# Autodesk Inventor assembly: PendulumAssembly
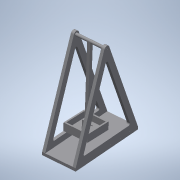
[picture p0: Inventor's stored thumbnail of the model, 180x180]
Saved by Autodesk Inventor 2020 (Build 240168000, 168)
## iProperties
Created: 2020-04-07
Part Number: PendulumAssembly
Document SubType Name: Assembly
Designer: gman
Author: gman
## Documents named in this file (5)
- C:\Users\gman\Desktop\CAD\Physics\PendulumAssembly.iam
- C:\Users\gman\Desktop\CAD\Physics\Outside.ipt
- C:\Users\gman\Desktop\CAD\Physics\PendulumHanger.ipt
- C:\Users\gman\Desktop\CAD\Physics\Base.ipt
- C:\Users\gman\Desktop\CAD\Physics\WeightBasket.ipt
## Components (5 placed, 4 different names)
1. Base:1 — Mate:1, Flush:1, Mate:2, Mate:3, Mate:4, Flush:2, Mate:8
2. Outside:1 — Mate:4, Flush:2, Rotational:1, Mate:8
3. Outside:2 — Flush:1, Mate:2, Mate:3, Flush:3
4. PendulumHanger:1 — Mate:5, Mate:6, Mate:7, Flush:3, Rotational:1
5. WeightBasket:1 — Mate:5, Mate:6, Mate:7
## Relationships (12: Mate 8, Flush 3, RevoluteJoint 1)
- Mate:1: Base:1
- Flush:1: Base:1 ↔ Outside:2
- Mate:2: Base:1 ↔ Outside:2
- Mate:3: Base:1 ↔ Outside:2
- Mate:4: Base:1 ↔ Outside:1
- Flush:2: Base:1 ↔ Outside:1
- Mate:5: PendulumHanger:1 ↔ WeightBasket:1
- Mate:6: PendulumHanger:1 ↔ WeightBasket:1
- Mate:7: PendulumHanger:1 ↔ WeightBasket:1
- Flush:3: Outside:2 ↔ PendulumHanger:1
- Rotational:1 [RevoluteJoint]: Outside:1 ↔ PendulumHanger:1
- Mate:8: Base:1 ↔ Outside:1
